# Autodesk Inventor assembly: full
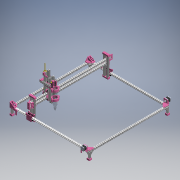
[picture p0: Inventor's stored thumbnail of the model, 180x180]
Saved by Autodesk Inventor 2019 (Build 230136000, 136)
## iProperties
Created: 2019-05-07
Part Number: full
Document SubType Name: Assembly
Designer: Alex Jones
Author: Alex Jones
## Documents named in this file (30)
- C:\Users\Alex Jones\Documents\Inventor\CNC\full.iam
- C:\Users\Alex Jones\Documents\Inventor\CNC\base.iam
- C:\Users\Alex Jones\Documents\Inventor\CNC\carriage.iam
- C:\Users\Alex Jones\Documents\Inventor\CNC\2020-1m.ipt
- C:\Users\Alex Jones\Documents\Inventor\CNC\cap.ipt
- C:\Users\Alex Jones\Documents\Inventor\CNC\2020-25cm.ipt
- C:\Users\Alex Jones\Documents\Inventor\CNC\double90.ipt
- C:\Users\Alex Jones\Documents\Inventor\CNC\bearingStandin.ipt
- C:\Users\Alex Jones\Documents\Inventor\CNC\couplerStandin.ipt
- C:\Users\Alex Jones\Documents\Inventor\CNC\nema17.ipt
- C:\Users\Alex Jones\Documents\Inventor\CNC\standinNut.ipt
- C:\Users\Alex Jones\Documents\Inventor\CNC\bed.iam
- C:\Users\Alex Jones\Documents\Inventor\CNC\roller.ipt
- C:\Users\Alex Jones\Documents\Inventor\CNC\yCarraige.ipt
- C:\Users\Alex Jones\Documents\Inventor\CNC\ZHolder.ipt
- C:\Users\Alex Jones\Documents\Inventor\CNC\threadedRodStandinShort.ipt
- C:\Users\Alex Jones\Documents\Inventor\CNC\Part3.ipt
- C:\Users\Alex Jones\Documents\Inventor\CNC\rollerHolderInnerZ.ipt
- C:\Users\Alex Jones\Documents\Inventor\CNC\Dremel.ipt
- C:\Users\Alex Jones\Documents\Inventor\CNC\DremelHolder.ipt
- C:\Users\Alex Jones\Documents\Inventor\CNC\dremelClamp.ipt
- C:\Users\Alex Jones\Documents\Inventor\CNC\ZNutHolder.ipt
- C:\Users\Alex Jones\Documents\Inventor\CNC\2020-125mm.ipt
- C:\Users\Alex Jones\Documents\Inventor\CNC\limitHolder.ipt
- C:\Users\Alex Jones\Documents\Inventor\CNC\nemaMountStock.ipt
- C:\Users\Alex Jones\Documents\Inventor\CNC\GT2_16T.ipt
- C:\Users\Alex Jones\Documents\Inventor\CNC\PULLEY 16T GT-2.ipt
- C:\Users\Alex Jones\Documents\Inventor\CNC\xTension.ipt
- C:\Users\Alex Jones\Documents\Inventor\CNC\limitHolderMirror.ipt
- C:\Users\Alex Jones\Documents\Inventor\CNC\double90andMotor.ipt
## Components (77 placed, 29 different names)
1. base:1 [sub-assembly] — Tangent:1, Tangent:2, Tangent:3, Tangent:4, Flush:40, Mate:145, Mate:146, Mate:151, Angle:17, Mate:154, Angle:18, Tangent:35, Mate:162, Mate:165, Angle:20, Mate:166, Mate:167, Mate:168, Mate:169, Mate:170
2. bed:1 [sub-assembly] — Flush:40
3. nemaMountStock:1 — Mate:145, Mate:146, Mate:147, Mate:148, Mate:149, Flush:72, Angle:20, Angle:21, Mate:171
4. nema17:4 — Mate:147, Mate:148, Mate:149, Mate:150
5. GT2_16T:1 — Mate:150
6. xTension:1 — Mate:151, Mate:152, Angle:17, Mate:156
7. PULLEY 16T GT-2:1 — Mate:152, Mate:156
8. xTension:2 — Mate:154, Mate:155, Angle:18
9. PULLEY 16T GT-2:2 — Mate:155
10. nemaMountStock:2 — Mate:162, Mate:165, Flush:72
11. nema17:5 — Mate:163
12. GT2_16T:2 — Mate:163
13. limitHolder:3 — Mate:166, Angle:21, Mate:167, Mate:171
14. limitHolderMirror:1 — Mate:168, Mate:169, Mate:170
15. GT2_16T:3 — Mate:172, Angle:22, Mate:173
16. nema17:6 — Mate:173, Angle:23, Mate:174, Mate:175
17. xTension:3 — Mate:181, Angle:24
18. PULLEY 16T GT-2:3
19. cap:5 — Mate:178, Mate:179, Mate:180, Mate:181
20. Part3:3 — Mate:182, Flush:74, Mate:183, Flush:75, Flush:76, Mate:185
21. 2020-125mm:2 — Mate:183, Flush:75, Flush:76
22. limitHolder:4 — Mate:192, Flush:80
23. limitHolderMirror:2 — Mate:190, Mate:191, Flush:79
24. cap:2 — Mate:12, Mate:13, Mate:14
25. cap:4 — Mate:18, Mate:19, Mate:20, Mate:21
26. 2020-25cm:3 — Mate:2, Mate:5, Flush:5, Flush:10, Flush:11, Mate:38
27. 2020-25cm:4 — Mate:4, Flush:5, Mate:12, Mate:13, Mate:14, Flush:10, Mate:18, Mate:19, Mate:20, Mate:37
28. carriage:2 [sub-assembly] — Tangent:1, Tangent:2, Tangent:3, Tangent:4, Mate:2, Mate:4, Mate:5, Mate:21, Angle:19, Tangent:36
29. cap:1 — Flush:9, Mate:9, Mate:10, Mate:11
30. cap:3 — Mate:15, Mate:16, Mate:17
31. 2020-25cm:1 — Mate:6, Flush:8, Mate:9, Mate:10, Mate:11, Flush:11, Mate:15, Mate:16, Mate:17, Mate:39, Mate:158
32. carriage:1 [sub-assembly] — Mate:6, Angle:19, Tangent:35, Mate:158, Mate:164, Tangent:36
33. 2020-25cm:2 — Flush:8, Flush:9, Mate:22, Mate:40, Mate:164
34. yCarraige:1 — Mate:80, Mate:81, Mate:85, Mate:86, Flush:43, Mate:87, Mate:88, Flush:44, Mate:89, Mate:114
35. yCarraige:2 — Mate:82, Mate:83, Mate:84, Mate:90, Flush:46, Flush:47, Mate:91, Flush:51, Mate:188, Mate:189
36. roller:4 — Tangent:11, Tangent:12, Mate:188
37. roller:3 — Tangent:13, Tangent:14, Mate:78, Mate:80, Mate:82, Mate:84, Mate:85
38. roller:2 — Tangent:15, Tangent:16, Mate:189
39. roller:1 — Tangent:17, Tangent:18, Mate:76, Mate:81, Mate:83
40. 2020-1m:5 — Mate:23, Flush:12, Flush:13, Mate:31, Mate:33, Flush:20, Flush:22, Tangent:11, Tangent:12, Tangent:13, Tangent:14, Angle:11, Angle:23, Flush:73, Mate:178, Mate:179, Mate:180
41. 2020-1m:6 — Mate:22, Mate:23, Flush:12, Flush:13, Mate:32, Mate:35, Tangent:15, Tangent:16, Tangent:17, Tangent:18, Mate:172, Angle:22, Angle:24, Mate:190, Mate:191, Flush:79, Mate:192, Flush:80
42. double90:1 — Mate:32, Mate:37, Flush:20, Flush:21
43. double90:2 — Mate:31, Mate:38, Flush:21
44. double90:3 — Mate:33, Mate:40, Flush:23, Flush:73
45. double90andMotor:1 — Mate:35, Mate:39, Flush:22, Flush:23, Mate:174, Mate:175
46. 2020-25cm:5 — Mate:88, Flush:44, Mate:89, Tangent:19, Tangent:20, Tangent:26, Tangent:27, Tangent:28
47. 2020-25cm:6 — Mate:86, Flush:43, Mate:87, Tangent:21, Tangent:22, Tangent:25, Tangent:30, Tangent:31, Tangent:32, Mate:115
48. 2020-25cm:7 — Mate:90, Flush:46, Mate:95, Mate:96, Mate:97, Mate:98, Flush:48, Flush:50, Mate:143, Flush:69, Flush:71
49. 2020-25cm:8 — Flush:47, Mate:91, Angle:8, Angle:9, Angle:10, Flush:48, Flush:53, Mate:142, Mate:144, Flush:70
50. bearingStandin:5 — Mate:95, Angle:8, Mate:96, Mate:99, Mate:100
51. bearingStandin:6 — Angle:9, Mate:97, Mate:98, Mate:102, Flush:53
52. nema17:3 — Mate:101, Angle:10, Flush:49, Mate:103, Flush:51, Mate:141
53. couplerStandin:3 — Mate:99, Mate:100, Mate:101, Flush:52
54. ZHolder:1 — Flush:49, Flush:50, Mate:141, Mate:142
55. threadedRodStandinShort:1 — Mate:102, Mate:103, Flush:52, Mate:104, Angle:12, Mate:186
56. standinNut:3 — Mate:104, Mate:136, Mate:137, Mate:140
57. roller:5 — Tangent:19, Tangent:20, Mate:105, Flush:78
58. roller:6 — Mate:106, Mate:121, Flush:78
59. roller:7 — Mate:106, Tangent:25, Mate:111, Mate:185
60. roller:8 — Tangent:21, Tangent:22, Mate:105, Mate:109
61. roller:9 — Tangent:26, Tangent:27, Mate:108, Mate:120
62. roller:10 — Tangent:28, Mate:107, Mate:119
63. roller:11 — Tangent:30, Tangent:31, Mate:108, Mate:112, Flush:77
64. roller:12 — Tangent:32, Mate:107, Mate:110, Mate:182, Flush:77, Mate:187
65. 2020-25cm:9 — Mate:114, Mate:115, Mate:122, Flush:55, Mate:124, Mate:125, Flush:56, Tangent:34, Mate:126, Mate:128, Flush:60, Mate:131, Flush:63
66. Part3:2 — Mate:119, Mate:120, Mate:121, Flush:64, Mate:134, Flush:65
67. rollerHolderInnerZ:1 — Mate:122, Flush:55, Mate:124, Flush:57, Mate:127, Mate:132, Mate:187
68. rollerHolderInnerZ:2 — Mate:125, Flush:56, Flush:57
69. Dremel:1 — Tangent:34, Angle:12, Mate:126, Mate:127
70. DremelHolder:1 — Flush:59, Mate:128, Flush:60, Flush:61, Mate:129, Angle:13
71. dremelClamp:1 — Flush:61, Mate:129, Angle:13, Mate:132, Mate:133
72. DremelHolder:2 — Mate:131, Flush:63, Mate:133
73. dremelClamp:2
74. 2020-125mm:1 — Flush:64, Mate:134, Flush:65, Flush:68, Mate:184
75. ZNutHolder:1 — Flush:68, Mate:140, Flush:74, Mate:184, Mate:186
76. limitHolder:1 — Mate:143, Flush:69, Flush:71
77. limitHolder:2 — Mate:144, Flush:70
## Relationships (220: Mate 133, Flush 45, Tangent 26, Angle 16)
- Tangent:1: base:1 ↔ carriage:2
- Tangent:2: base:1 ↔ carriage:2
- Tangent:3: base:1 ↔ carriage:2
- Tangent:4: base:1 ↔ carriage:2
- Mate:2 (-10 mm): 2020-25cm:3 ↔ carriage:2
- Mate:4 (-10 mm): 2020-25cm:4 ↔ carriage:2
- Mate:5: 2020-25cm:3 ↔ carriage:2
- Flush:5: 2020-25cm:3 ↔ 2020-25cm:4
- Mate:6: 2020-25cm:1 ↔ carriage:1
- Flush:8: 2020-25cm:1 ↔ 2020-25cm:2
- Flush:9: cap:1 ↔ 2020-25cm:2
- Mate:9: cap:1 ↔ 2020-25cm:1
- Mate:10: cap:1 ↔ 2020-25cm:1
- Mate:11: cap:1 ↔ 2020-25cm:1
- Mate:12: cap:2 ↔ 2020-25cm:4
- Mate:13: cap:2 ↔ 2020-25cm:4
- Mate:14: cap:2 ↔ 2020-25cm:4
- Flush:10: 2020-25cm:3 ↔ 2020-25cm:4
- Flush:11: 2020-25cm:3 ↔ 2020-25cm:1
- Mate:15: cap:3 ↔ 2020-25cm:1
- Mate:16: cap:3 ↔ 2020-25cm:1
- Mate:17: cap:3 ↔ 2020-25cm:1
- Mate:18: cap:4 ↔ 2020-25cm:4
- Mate:19: cap:4 ↔ 2020-25cm:4
- Mate:20: cap:4 ↔ 2020-25cm:4
- Mate:21 (1.27 mm): cap:4 ↔ carriage:2
- Mate:22: 2020-25cm:2 ↔ 2020-1m:6
- Mate:23 (20 mm): 2020-1m:5 ↔ 2020-1m:6
- Flush:12: 2020-1m:5 ↔ 2020-1m:6
- Flush:13: 2020-1m:5 ↔ 2020-1m:6
- Mate:31: 2020-1m:5 ↔ double90:2
- Mate:32: 2020-1m:6 ↔ double90:1
- Mate:33: 2020-1m:5 ↔ double90:3
- Mate:35: 2020-1m:6 ↔ double90andMotor:1
- Mate:37: 2020-25cm:4 ↔ double90:1
- Flush:20: 2020-1m:5 ↔ double90:1
- Mate:38: 2020-25cm:3 ↔ double90:2
- Flush:21: double90:1 ↔ double90:2
- Mate:39: 2020-25cm:1 ↔ double90andMotor:1
- Flush:22: 2020-1m:5 ↔ double90andMotor:1
- Mate:40: 2020-25cm:2 ↔ double90:3
- Flush:23: double90:3 ↔ double90andMotor:1
- Flush:40: base:1 ↔ bed:1
- Tangent:11: roller:4 ↔ 2020-1m:5
- Tangent:12: roller:4 ↔ 2020-1m:5
- Tangent:13: roller:3 ↔ 2020-1m:5
- Tangent:14: roller:3 ↔ 2020-1m:5
- Tangent:15: roller:2 ↔ 2020-1m:6
- Tangent:16: roller:2 ↔ 2020-1m:6
- Tangent:17: roller:1 ↔ 2020-1m:6
- Tangent:18: roller:1 ↔ 2020-1m:6
- Mate:76: roller:1
- Mate:78: roller:3
- Angle:6 (0 deg)
- Mate:80: yCarraige:1 ↔ roller:3
- Mate:81: yCarraige:1 ↔ roller:1
- Mate:82: yCarraige:2 ↔ roller:3
- Mate:83: yCarraige:2 ↔ roller:1
- Mate:84 (6 mm): yCarraige:2 ↔ roller:3
- Mate:85 (6 mm): yCarraige:1 ↔ roller:3
- Mate:86: yCarraige:1 ↔ 2020-25cm:6
- Flush:43: yCarraige:1 ↔ 2020-25cm:6
- Mate:87 (-10 mm): yCarraige:1 ↔ 2020-25cm:6
- Mate:88: yCarraige:1 ↔ 2020-25cm:5
- Flush:44: yCarraige:1 ↔ 2020-25cm:5
- Mate:89 (-10 mm): yCarraige:1 ↔ 2020-25cm:5
- Mate:90: yCarraige:2 ↔ 2020-25cm:7
- Flush:46: yCarraige:2 ↔ 2020-25cm:7
- Flush:47: yCarraige:2 ↔ 2020-25cm:8
- Mate:91: yCarraige:2 ↔ 2020-25cm:8
- Mate:95: 2020-25cm:7 ↔ bearingStandin:5
- Angle:8 (0 deg): 2020-25cm:8 ↔ bearingStandin:5
- Mate:96 (-10 mm): 2020-25cm:7 ↔ bearingStandin:5
- Angle:9 (0 deg): 2020-25cm:8 ↔ bearingStandin:6
- Mate:97: 2020-25cm:7 ↔ bearingStandin:6
- Mate:98 (-10 mm): 2020-25cm:7 ↔ bearingStandin:6
- Mate:99: bearingStandin:5 ↔ couplerStandin:3
- Mate:100: bearingStandin:5 ↔ couplerStandin:3
- Mate:101: nema17:3 ↔ couplerStandin:3
- Angle:10 (45 deg): 2020-25cm:8 ↔ nema17:3
- Flush:48: 2020-25cm:7 ↔ 2020-25cm:8
- Flush:49: nema17:3 ↔ ZHolder:1
- Flush:50: 2020-25cm:7 ↔ ZHolder:1
- Mate:102: bearingStandin:6 ↔ threadedRodStandinShort:1
- Mate:103: nema17:3 ↔ threadedRodStandinShort:1
- Flush:51: yCarraige:2 ↔ nema17:3
- Flush:52 (-12 mm): couplerStandin:3 ↔ threadedRodStandinShort:1
- Flush:53 (15 mm): 2020-25cm:8 ↔ bearingStandin:6
- Mate:104: threadedRodStandinShort:1 ↔ standinNut:3
- Tangent:19: 2020-25cm:5 ↔ roller:5
- Tangent:20: 2020-25cm:5 ↔ roller:5
- Tangent:21: 2020-25cm:6 ↔ roller:8
- Tangent:22: 2020-25cm:6 ↔ roller:8
- Mate:105: roller:5 ↔ roller:8
- Mate:106: roller:6 ↔ roller:7
- Tangent:25: 2020-25cm:6 ↔ roller:7
- Tangent:26: 2020-25cm:5 ↔ roller:9
- Tangent:27: 2020-25cm:5 ↔ roller:9
- Tangent:28: 2020-25cm:5 ↔ roller:10
- Tangent:30: 2020-25cm:6 ↔ roller:11
- Tangent:31: 2020-25cm:6 ↔ roller:11
- Tangent:32: 2020-25cm:6 ↔ roller:12
- Mate:107: roller:10 ↔ roller:12
- Mate:108: roller:9 ↔ roller:11
- Mate:109: roller:8
- Mate:110: roller:12
- Mate:111: roller:7
- Mate:112: roller:11
- Angle:11 (0 deg): 2020-1m:5
- Mate:113 (25 mm)
- Mate:114: yCarraige:1 ↔ 2020-25cm:9
- Mate:115 (1 mm): 2020-25cm:6 ↔ 2020-25cm:9
- Mate:119: roller:10 ↔ Part3:2
- Mate:120 (6 mm): roller:9 ↔ Part3:2
- Mate:121: roller:6 ↔ Part3:2
- Mate:122: 2020-25cm:9 ↔ rollerHolderInnerZ:1
- Flush:55: 2020-25cm:9 ↔ rollerHolderInnerZ:1
- Mate:124 (-10 mm): 2020-25cm:9 ↔ rollerHolderInnerZ:1
- Mate:125: 2020-25cm:9 ↔ rollerHolderInnerZ:2
- Flush:56: 2020-25cm:9 ↔ rollerHolderInnerZ:2
- Flush:57: rollerHolderInnerZ:1 ↔ rollerHolderInnerZ:2
- Tangent:34 (12.7 mm): 2020-25cm:9 ↔ Dremel:1
- Angle:12 (180 deg): threadedRodStandinShort:1 ↔ Dremel:1
- Mate:126 (-10 mm): 2020-25cm:9 ↔ Dremel:1
- Mate:127: rollerHolderInnerZ:1 ↔ Dremel:1
- Flush:59: DremelHolder:1
- Mate:128: 2020-25cm:9 ↔ DremelHolder:1
- Flush:60: 2020-25cm:9 ↔ DremelHolder:1
- Flush:61: DremelHolder:1 ↔ dremelClamp:1
- Mate:129: DremelHolder:1 ↔ dremelClamp:1
- Angle:13 (180 deg): DremelHolder:1 ↔ dremelClamp:1
- [Flush]: DremelHolder:2 ↔ dremelClamp:2
- [Mate]: DremelHolder:2 ↔ dremelClamp:2
- [Angle] (180 deg): DremelHolder:2 ↔ dremelClamp:2
- Mate:131: 2020-25cm:9 ↔ DremelHolder:2
- Flush:63: 2020-25cm:9 ↔ DremelHolder:2
- Mate:132: rollerHolderInnerZ:1 ↔ dremelClamp:1
- Mate:133 (76.2 mm): dremelClamp:1 ↔ DremelHolder:2
- Flush:64: Part3:2 ↔ 2020-125mm:1
- Mate:134: Part3:2 ↔ 2020-125mm:1
- Flush:65: Part3:2 ↔ 2020-125mm:1
- Flush:68: 2020-125mm:1 ↔ ZNutHolder:1
- Mate:136: standinNut:3
- Mate:137: standinNut:3
- Mate:138
- Mate:139
- Mate:140: standinNut:3 ↔ ZNutHolder:1
- Mate:141: nema17:3 ↔ ZHolder:1
- Mate:142: 2020-25cm:8 ↔ ZHolder:1
- Mate:143: 2020-25cm:7 ↔ limitHolder:1
- Flush:69: 2020-25cm:7 ↔ limitHolder:1
- Mate:144: 2020-25cm:8 ↔ limitHolder:2
- Flush:70: 2020-25cm:8 ↔ limitHolder:2
- Flush:71: 2020-25cm:7 ↔ limitHolder:1
- Mate:145: base:1 ↔ nemaMountStock:1
- Mate:146 (-10 mm): base:1 ↔ nemaMountStock:1
- Mate:147: nemaMountStock:1 ↔ nema17:4
- Mate:148: nemaMountStock:1 ↔ nema17:4
- Mate:149: nemaMountStock:1 ↔ nema17:4
- Mate:150: nema17:4 ↔ GT2_16T:1
- Mate:151: base:1 ↔ xTension:1
- Mate:152: xTension:1 ↔ PULLEY 16T GT-2:1
- Angle:17 (0 deg): base:1 ↔ xTension:1
- [Mate]: xTension:2 ↔ PULLEY 16T GT-2:2
- Mate:154: base:1 ↔ xTension:2
- Mate:155 (0.75 mm): xTension:2 ↔ PULLEY 16T GT-2:2
- Mate:156 (0.75 mm): xTension:1 ↔ PULLEY 16T GT-2:1
- Angle:18 (0 deg): base:1 ↔ xTension:2
- Angle:19 (0 deg): carriage:2 ↔ carriage:1
- Tangent:35: base:1 ↔ carriage:1
- Mate:158 (-10 mm): 2020-25cm:1 ↔ carriage:1
- [Mate]: nemaMountStock:2 ↔ nema17:5
- [Mate]: nemaMountStock:2 ↔ nema17:5
- [Mate]: nemaMountStock:2 ↔ nema17:5
- Mate:162: base:1 ↔ nemaMountStock:2
- Mate:163: nema17:5 ↔ GT2_16T:2
- Mate:164 (-10 mm): carriage:1 ↔ 2020-25cm:2
- Tangent:36: carriage:2 ↔ carriage:1
- Mate:165 (-10 mm): base:1 ↔ nemaMountStock:2
- Flush:72: nemaMountStock:1 ↔ nemaMountStock:2
- Angle:20 (0 deg): base:1 ↔ nemaMountStock:1
- Mate:166: base:1 ↔ limitHolder:3
- Angle:21 (0 deg): nemaMountStock:1 ↔ limitHolder:3
- Mate:167 (-10 mm): base:1 ↔ limitHolder:3
- Mate:168: base:1 ↔ limitHolderMirror:1
- Mate:169 (-10 mm): base:1 ↔ limitHolderMirror:1
- Mate:170: base:1 ↔ limitHolderMirror:1
- Mate:171: nemaMountStock:1 ↔ limitHolder:3
- Mate:172 (10 mm): GT2_16T:3 ↔ 2020-1m:6
- Angle:22 (0 deg): GT2_16T:3 ↔ 2020-1m:6
- Mate:173: GT2_16T:3 ↔ nema17:6
- Angle:23 (0 deg): nema17:6 ↔ 2020-1m:5
- Flush:73: 2020-1m:5 ↔ double90:3
- Mate:174: nema17:6 ↔ double90andMotor:1
- Mate:175: nema17:6 ↔ double90andMotor:1
- [Mate]: xTension:3 ↔ PULLEY 16T GT-2:3
- [Mate] (0.75 mm): xTension:3 ↔ PULLEY 16T GT-2:3
- Mate:178: cap:5 ↔ 2020-1m:5
- Mate:179: cap:5 ↔ 2020-1m:5
- Mate:180: cap:5 ↔ 2020-1m:5
- Mate:181: xTension:3 ↔ cap:5
- Angle:24 (0 deg): xTension:3 ↔ 2020-1m:6
- Mate:182: Part3:3 ↔ roller:12
- Flush:74: Part3:3 ↔ ZNutHolder:1
- Mate:183: Part3:3 ↔ 2020-125mm:2
- Flush:75: Part3:3 ↔ 2020-125mm:2
- Flush:76: Part3:3 ↔ 2020-125mm:2
- Mate:184: 2020-125mm:1 ↔ ZNutHolder:1
- Flush:77: roller:11 ↔ roller:12
- Flush:78: roller:5 ↔ roller:6
- Mate:185: Part3:3 ↔ roller:7
- Mate:186: threadedRodStandinShort:1 ↔ ZNutHolder:1
- Mate:187: roller:12 ↔ rollerHolderInnerZ:1
- Mate:188: yCarraige:2 ↔ roller:4
- Mate:189: yCarraige:2 ↔ roller:2
- Mate:190: limitHolderMirror:2 ↔ 2020-1m:6
- Mate:191: limitHolderMirror:2 ↔ 2020-1m:6
- Flush:79: limitHolderMirror:2 ↔ 2020-1m:6
- Mate:192: limitHolder:4 ↔ 2020-1m:6
- Flush:80: limitHolder:4 ↔ 2020-1m:6
## Named parameters: d327_d324 = 0 mm, d328_d325 = 0 mm, d329_d326 = 180 deg, d374_d372 = 0 mm, d383_d363 = 0 mm, d384_d364 = 0 mm, d385_d365 = 0 mm, d416_d377 = 0.75 mm, d417_d372 = 0 mm
